# Autodesk Inventor assembly: folivora
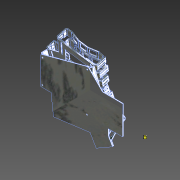
[picture p0: Inventor's stored thumbnail of the model, 180x180]
Saved by Autodesk Inventor 2018 (Build 220112000, 112)
## iProperties
Created: 2018-05-16
Part Number: folivora
Material: 一般
Document SubType Name: Assembly
Designer: NaMACHAN
Mass: 281.35 g
Surface Area: 1214.73 cm^2
Volume: 104.204 cm^3
Density: 2.7 g/cm^3
Author: NaMACHAN
## Documents named in this file (11)
- C:\Users\NaMACHAN\Dropbox\Project\original\folivora\inventor\folivora.iam
- C:\Users\NaMACHAN\Dropbox\Project\original\folivora\inventor\frame.ipt
- C:\Users\NaMACHAN\Dropbox\Project\original\folivora\inventor\ThumbPlate.ipt
- C:\Users\NaMACHAN\Dropbox\Project\original\folivora\inventor\Part6.ipt
- C:\Users\NaMACHAN\Dropbox\Project\original\folivora\inventor\baseframe.ipt
- C:\Users\NaMACHAN\Dropbox\Project\original\folivora\inventor\keyplate4.ipt
- C:\Users\NaMACHAN\Dropbox\Project\original\folivora\inventor\keyplate5.ipt
- C:\Users\NaMACHAN\Dropbox\Project\original\folivora\inventor\keyplate3.ipt
- C:\Users\NaMACHAN\Dropbox\Project\original\folivora\inventor\keyL_large.ipt
- C:\Users\NaMACHAN\Dropbox\Project\original\folivora\inventor\keyL_medium.ipt
- C:\Users\NaMACHAN\Dropbox\Project\original\folivora\inventor\keyL_small.ipt
## Components (23 placed, 10 different names)
1. frame:1 — フラッシュ:27, メイト:1, メイト:31, メイト:32, メイト:33, メイト:34, メイト:35, メイト:36, メイト:37, メイト:38, メイト:39, メイト:40, メイト:41, メイト:42, メイト:43, メイト:44, メイト:45, メイト:46, メイト:47, メイト:48, フラッシュ:43
2. ThumbPlate:1 — フラッシュ:28, メイト:2, フラッシュ:30
3. ThumbPlate:2 — メイト:3, フラッシュ:29, フラッシュ:31
4. Part6:1 — フラッシュ:27
5. baseframe:1 — メイト:1, フラッシュ:28, メイト:2, メイト:3, フラッシュ:29, フラッシュ:30, フラッシュ:31
6. keyplate4:1 — メイト:18, メイト:19, メイト:20, メイト:21, メイト:22, 角度:5
7. keyplate5:1 — メイト:4, メイト:5, メイト:6, メイト:7, メイト:8, メイト:9, 角度:4, 角度:6
8. keyplate3:1 — フラッシュ:39, メイト:23, メイト:24, メイト:25, メイト:26, 角度:2, 角度:3
9. keyL_large:1 — フラッシュ:39, メイト:23, メイト:24, フラッシュ:40
10. keyL_medium:1 — フラッシュ:33, メイト:10, メイト:11, フラッシュ:34, メイト:34
11. keyL_small:1 — メイト:4, メイト:5, メイト:6, フラッシュ:32, メイト:8, メイト:43, メイト:44, フラッシュ:43
12. keyL_small:2 — フラッシュ:32, メイト:7, メイト:9, メイト:33
13. keyplate5:2 — フラッシュ:33, メイト:10, メイト:11, メイト:12, メイト:13, 角度:4, 角度:5
14. keyL_medium:2 — フラッシュ:34, メイト:12, メイト:13, メイト:45, メイト:46
15. keyL_medium:3
16. keyplate5:3 — 角度:2, 角度:6
17. keyL_medium:4 — メイト:32, メイト:41, メイト:42
18. keyL_medium:5 — メイト:18, メイト:19, メイト:20, フラッシュ:37, フラッシュ:38, メイト:35, メイト:47, メイト:48
19. keyL_medium:6 — フラッシュ:37, メイト:21, メイト:22, フラッシュ:38
20. keyL_large:2 — フラッシュ:40, メイト:25, メイト:26, メイト:36, メイト:39, メイト:40
21. keyplate3:2 — 角度:3
22. keyL_large:3
23. keyL_large:4 — メイト:31, メイト:37, メイト:38
## Relationships (70: Mate 48, Flush 17, Angle 5)
- フラッシュ:27 [Flush]: frame:1 ↔ Part6:1
- メイト:1 [Mate]: frame:1 ↔ baseframe:1
- フラッシュ:28 [Flush]: ThumbPlate:1 ↔ baseframe:1
- メイト:2 [Mate]: ThumbPlate:1 ↔ baseframe:1
- メイト:3 [Mate]: ThumbPlate:2 ↔ baseframe:1
- フラッシュ:29 [Flush]: ThumbPlate:2 ↔ baseframe:1
- フラッシュ:30 [Flush]: ThumbPlate:1 ↔ baseframe:1
- フラッシュ:31 [Flush]: ThumbPlate:2 ↔ baseframe:1
- メイト:4 [Mate]: keyplate5:1 ↔ keyL_small:1
- メイト:5 [Mate]: keyplate5:1 ↔ keyL_small:1
- メイト:6 [Mate]: keyplate5:1 ↔ keyL_small:1
- フラッシュ:32 [Flush]: keyL_small:1 ↔ keyL_small:2
- メイト:7 [Mate]: keyplate5:1 ↔ keyL_small:2
- メイト:8 [Mate]: keyplate5:1 ↔ keyL_small:1
- メイト:9 [Mate]: keyplate5:1 ↔ keyL_small:2
- フラッシュ:33 [Flush]: keyL_medium:1 ↔ keyplate5:2
- メイト:10 [Mate]: keyL_medium:1 ↔ keyplate5:2
- メイト:11 [Mate] (1.5 mm): keyL_medium:1 ↔ keyplate5:2
- フラッシュ:34 [Flush]: keyL_medium:1 ↔ keyL_medium:2
- メイト:12 [Mate]: keyplate5:2 ↔ keyL_medium:2
- メイト:13 [Mate] (1.5 mm): keyplate5:2 ↔ keyL_medium:2
- [Flush]: keyL_medium:3 ↔ keyplate5:3
- [Mate]: keyL_medium:3 ↔ keyplate5:3
- [Mate] (1.5 mm): keyL_medium:3 ↔ keyplate5:3
- [Flush]: keyL_medium:3 ↔ keyL_medium:4
- [Mate]: keyplate5:3 ↔ keyL_medium:4
- [Mate] (1.5 mm): keyplate5:3 ↔ keyL_medium:4
- メイト:18 [Mate]: keyplate4:1 ↔ keyL_medium:5
- メイト:19 [Mate]: keyplate4:1 ↔ keyL_medium:5
- メイト:20 [Mate]: keyplate4:1 ↔ keyL_medium:5
- フラッシュ:37 [Flush]: keyL_medium:5 ↔ keyL_medium:6
- メイト:21 [Mate]: keyplate4:1 ↔ keyL_medium:6
- メイト:22 [Mate] (1.5 mm): keyplate4:1 ↔ keyL_medium:6
- フラッシュ:38 [Flush]: keyL_medium:5 ↔ keyL_medium:6
- フラッシュ:39 [Flush]: keyplate3:1 ↔ keyL_large:1
- メイト:23 [Mate]: keyplate3:1 ↔ keyL_large:1
- メイト:24 [Mate] (1.5 mm): keyplate3:1 ↔ keyL_large:1
- フラッシュ:40 [Flush]: keyL_large:1 ↔ keyL_large:2
- メイト:25 [Mate]: keyplate3:1 ↔ keyL_large:2
- メイト:26 [Mate] (1.5 mm): keyplate3:1 ↔ keyL_large:2
- [Flush]: keyplate3:2 ↔ keyL_large:3
- [Mate]: keyplate3:2 ↔ keyL_large:3
- [Mate] (1.5 mm): keyplate3:2 ↔ keyL_large:3
- [Flush]: keyL_large:3 ↔ keyL_large:4
- [Mate]: keyplate3:2 ↔ keyL_large:4
- [Mate] (1.5 mm): keyplate3:2 ↔ keyL_large:4
- メイト:31 [Mate]: frame:1 ↔ keyL_large:4
- メイト:32 [Mate]: frame:1 ↔ keyL_medium:4
- メイト:33 [Mate]: frame:1 ↔ keyL_small:2
- メイト:34 [Mate]: frame:1 ↔ keyL_medium:1
- メイト:35 [Mate]: frame:1 ↔ keyL_medium:5
- メイト:36 [Mate]: frame:1 ↔ keyL_large:2
- メイト:37 [Mate] (-8 mm): frame:1 ↔ keyL_large:4
- メイト:38 [Mate] (-20 mm): frame:1 ↔ keyL_large:4
- メイト:39 [Mate] (-30 mm): frame:1 ↔ keyL_large:2
- メイト:40 [Mate] (-20 mm): frame:1 ↔ keyL_large:2
- メイト:41 [Mate] (-52 mm): frame:1 ↔ keyL_medium:4
- メイト:42 [Mate] (-20 mm): frame:1 ↔ keyL_medium:4
- メイト:43 [Mate] (-76 mm): frame:1 ↔ keyL_small:1
- メイト:44 [Mate] (-20 mm): frame:1 ↔ keyL_small:1
- メイト:45 [Mate] (-20 mm): frame:1 ↔ keyL_medium:2
- メイト:46 [Mate] (-96 mm): frame:1 ↔ keyL_medium:2
- メイト:47 [Mate] (-20 mm): frame:1 ↔ keyL_medium:5
- メイト:48 [Mate] (-120 mm): frame:1 ↔ keyL_medium:5
- 角度:2 [Angle] (4 deg): keyplate3:1 ↔ keyplate5:3
- 角度:3 [Angle] (4 deg): keyplate3:1 ↔ keyplate3:2
- 角度:4 [Angle] (4 deg): keyplate5:1 ↔ keyplate5:2
- 角度:5 [Angle] (4 deg): keyplate4:1 ↔ keyplate5:2
- フラッシュ:43 [Flush]: frame:1 ↔ keyL_small:1
- 角度:6 [Angle] (4 deg): keyplate5:1 ↔ keyplate5:3
## Named parameters: d209_d203 = 0 mm, d210_d204 = 0 mm, d211_d205 = 1.5 mm, d212_d206 = 0 mm, d213_d207 = 0 mm, d214_d208 = 1.5 mm, d229_d223 = 0 mm, d230_d224 = 0 mm, d231_d225 = 1.5 mm, d232_d226 = 0 mm, d233_d227 = 0 mm, d234_d228 = 1.5 mm
